# Autodesk Inventor assembly: Main_Assembly
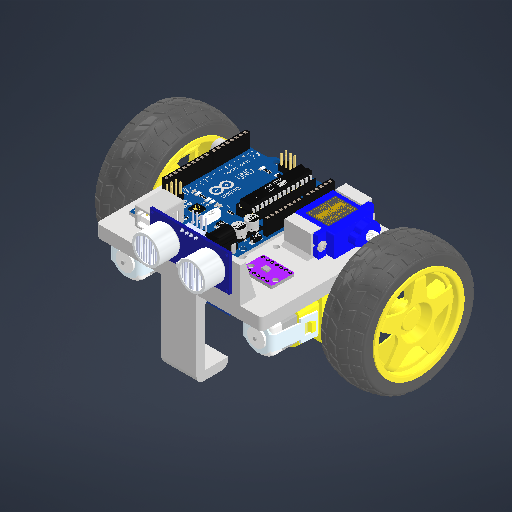
[picture p0: Inventor's stored thumbnail of the model, 512x512]
Saved by Autodesk Inventor 2026.1 (Build 301233020, 233B)
## iProperties
Created: 2025-10-16
Part Number: Main_Assembly
Document SubType Name: Assembly
Designer: Garfieldcmix
Author: Garfieldcmix
## Documents named in this file (11)
- C:\Users\Garfieldcmix\git\KMITL-ComPro-Group-Work\models\auto-robot\Auto_Robot.iam
- C:\Users\Garfieldcmix\git\KMITL-ComPro-Group-Work\models\auto-robot\Chassis.ipt
- C:\Users\Garfieldcmix\git\KMITL-ComPro-Group-Work\models\auto-robot\Front_Skit_Plate.ipt
- C:\Users\Garfieldcmix\git\KMITL-ComPro-Group-Work\models\auto-robot\Motor_Holder.ipt
- C:\Users\Garfieldcmix\git\KMITL-ComPro-Group-Work\models\auto-robot\components\DC Motor TT.ipt
- C:\Users\Garfieldcmix\git\KMITL-ComPro-Group-Work\models\auto-robot\components\SG90 servo motor.ipt
- C:\Users\Garfieldcmix\git\KMITL-ComPro-Group-Work\models\auto-robot\components\Arudino Uno.ipt
- C:\Users\Garfieldcmix\git\KMITL-ComPro-Group-Work\models\auto-robot\components\Wheel.ipt
- C:\Users\Garfieldcmix\git\KMITL-ComPro-Group-Work\models\auto-robot\components\HC-SR04.ipt
- C:\Users\Garfieldcmix\git\KMITL-ComPro-Group-Work\models\auto-robot\components\BMI 160.ipt
- C:\Users\Garfieldcmix\git\KMITL-ComPro-Group-Work\models\auto-robot\components\L298N.ipt
## Components (13 placed, 10 different names)
1. Chassis:1 — Mate:1, Mate:2, Mate:3, Mate:4, Mate:5, Mate:6, Mate:7, Mate:8, Mate:9, Mate:10, Mate:13, Mate:16, Mate:17, Mate:18, Mate:19, Tangent:1, Mate:20, Mate:25, Flush:1, Mate:26, Mate:27, Mate:28, Mate:29
2. Front_Skit_Plate:1 — Mate:1, Mate:2, Mate:3
3. Motor_Holder:1 — Mate:4, Mate:5, Mate:6, Mate:11, Mate:12
4. Motor_Holder:2 — Mate:7, Mate:8, Mate:9, Mate:14, Mate:15
5. DC Motor TT:1 — Mate:10, Mate:11, Mate:12, Mate:21, Mate:22
6. DC Motor TT:2 — Mate:13, Mate:14, Mate:15, Mate:23, Mate:24
7. SG90 servo motor:1 — Mate:16, Mate:17, Mate:18
8. Arudino Uno:1 — Mate:19, Tangent:1, Mate:20
9. Wheel:1 — Mate:21, Mate:22
10. Wheel:2 — Mate:23, Mate:24
11. HC-SR04:1 — Mate:25, Flush:1
12. BMI 160:1 — Mate:26
13. L298N:1 — Mate:27, Mate:28, Mate:29
## Relationships (31: Mate 29, Tangent 1, Flush 1)
- Mate:1: Chassis:1 ↔ Front_Skit_Plate:1
- Mate:2: Chassis:1 ↔ Front_Skit_Plate:1
- Mate:3: Chassis:1 ↔ Front_Skit_Plate:1
- Mate:4: Chassis:1 ↔ Motor_Holder:1
- Mate:5: Chassis:1 ↔ Motor_Holder:1
- Mate:6: Chassis:1 ↔ Motor_Holder:1
- Mate:7: Chassis:1 ↔ Motor_Holder:2
- Mate:8: Chassis:1 ↔ Motor_Holder:2
- Mate:9: Chassis:1 ↔ Motor_Holder:2
- Mate:10: Chassis:1 ↔ DC Motor TT:1
- Mate:11: Motor_Holder:1 ↔ DC Motor TT:1
- Mate:12: Motor_Holder:1 ↔ DC Motor TT:1
- Mate:13: Chassis:1 ↔ DC Motor TT:2
- Mate:14: Motor_Holder:2 ↔ DC Motor TT:2
- Mate:15: Motor_Holder:2 ↔ DC Motor TT:2
- Mate:16: Chassis:1 ↔ SG90 servo motor:1
- Mate:17: Chassis:1 ↔ SG90 servo motor:1
- Mate:18: Chassis:1 ↔ SG90 servo motor:1
- Mate:19: Chassis:1 ↔ Arudino Uno:1
- Tangent:1: Chassis:1 ↔ Arudino Uno:1
- Mate:20: Chassis:1 ↔ Arudino Uno:1
- Mate:21: DC Motor TT:1 ↔ Wheel:1
- Mate:22: DC Motor TT:1 ↔ Wheel:1
- Mate:23: DC Motor TT:2 ↔ Wheel:2
- Mate:24: DC Motor TT:2 ↔ Wheel:2
- Mate:25: Chassis:1 ↔ HC-SR04:1
- Flush:1 (-5 mm): Chassis:1 ↔ HC-SR04:1
- Mate:26: Chassis:1 ↔ BMI 160:1
- Mate:27 (3 mm): Chassis:1 ↔ L298N:1
- Mate:28: Chassis:1 ↔ L298N:1
- Mate:29: Chassis:1 ↔ L298N:1
